# Autodesk Inventor assembly: FULL FINGE6
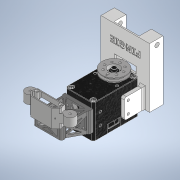
[picture p0: Inventor's stored thumbnail of the model, 180x180]
Saved by Autodesk Inventor 2021 (Build 250183000, 183)
## iProperties
Created: 2022-10-03
Part Number: FULL FINGE6
Document SubType Name: Assembly
Designer: ereg140
Author: ereg140
## Documents named in this file (6)
- \\files.auckland.ac.nz\myhome\Documents\GitHub\hand\FULL FINGE6.iam
- \\files.auckland.ac.nz\myhome\Documents\GitHub\hand\XM430 Motor\XM430-Working-Shaft.iam
- \\files.auckland.ac.nz\myhome\Documents\GitHub\hand\Phalalnge5_palm_dynamixel.ipt
- \\files.auckland.ac.nz\myhome\Documents\GitHub\hand\Pully_smlaller.ipt
- \\files.auckland.ac.nz\myhome\Documents\GitHub\hand\Dovetail\dovetail_female_Dyna_Mount.ipt
- \\files.auckland.ac.nz\myhome\Documents\GitHub\hand\Dynamixel_Palm_Bracket_2.ipt
## Components (5 placed, 5 different names)
1. XM430-Working-Shaft:1 [sub-assembly] — Angle:1, Rigid:4, Mate:1, Mate:2, Slider:1, Rigid:7
2. Phalalnge5_palm_dynamixel:1 — Rigid:6
3. Pully_smlaller:1 — Rigid:4
4. dovetail_female_Dyna_Mount:1 — Mate:1, Mate:2, Slider:1
5. Dynamixel_Palm_Bracket_2:1 — Rigid:6, Rigid:7
## Relationships (7: WeldJoint 3, Mate 2, Angle 1, TranslationJoint 1)
- Angle:1 (0 deg): XM430-Working-Shaft:1
- Rigid:4 [WeldJoint]: XM430-Working-Shaft:1 ↔ Pully_smlaller:1
- Mate:1: XM430-Working-Shaft:1 ↔ dovetail_female_Dyna_Mount:1
- Mate:2: XM430-Working-Shaft:1 ↔ dovetail_female_Dyna_Mount:1
- Slider:1 [TranslationJoint]: XM430-Working-Shaft:1 ↔ dovetail_female_Dyna_Mount:1
- Rigid:6 [WeldJoint]: Phalalnge5_palm_dynamixel:1 ↔ Dynamixel_Palm_Bracket_2:1
- Rigid:7 [WeldJoint]: XM430-Working-Shaft:1 ↔ Dynamixel_Palm_Bracket_2:1
## Named parameters: sa_0 = 30000
note: some values were not read from the file. Shown as the stored number, unit unknown: "sa_0".
